# Autodesk Inventor assembly: 2x20ExtraTallHeader
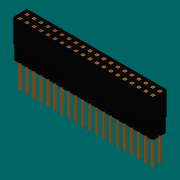
[picture p0: Inventor's stored thumbnail of the model, 180x180]
Saved by Autodesk Inventor 2016 SP1 (Build 200210100, 210)
## iProperties
Created: 2016-04-06
Part Number: 2x20ExtraTallHeader
Document SubType Name: Assembly
Designer: sawai
Author: sawai
## Documents named in this file (2)
- C:\Users\sawai\OneDrive\projects\mppcInterface\cad\connector\2.54Header\piExtraTall\2x20ExtraTallHeader.iam
- C:\Users\sawai\OneDrive\projects\mppcInterface\cad\connector\2.54Header\piExtraTall\extraTallPin.iam
## Components (40 placed, 1 different names)
1. extraTallPin:1 [sub-assembly]
2. extraTallPin:2 [sub-assembly]
3. extraTallPin:3 [sub-assembly]
4. extraTallPin:4 [sub-assembly]
5. extraTallPin:5 [sub-assembly]
6. extraTallPin:6 [sub-assembly]
7. extraTallPin:7 [sub-assembly]
8. extraTallPin:8 [sub-assembly]
9. extraTallPin:9 [sub-assembly]
10. extraTallPin:10 [sub-assembly]
11. extraTallPin:11 [sub-assembly]
12. extraTallPin:12 [sub-assembly]
13. extraTallPin:13 [sub-assembly]
14. extraTallPin:14 [sub-assembly]
15. extraTallPin:15 [sub-assembly]
16. extraTallPin:16 [sub-assembly]
17. extraTallPin:17 [sub-assembly]
18. extraTallPin:18 [sub-assembly]
19. extraTallPin:19 [sub-assembly]
20. extraTallPin:20 [sub-assembly]
21. extraTallPin:21 [sub-assembly]
22. extraTallPin:22 [sub-assembly]
23. extraTallPin:23 [sub-assembly]
24. extraTallPin:24 [sub-assembly]
25. extraTallPin:25 [sub-assembly]
26. extraTallPin:26 [sub-assembly]
27. extraTallPin:27 [sub-assembly]
28. extraTallPin:28 [sub-assembly]
29. extraTallPin:29 [sub-assembly]
30. extraTallPin:30 [sub-assembly]
31. extraTallPin:31 [sub-assembly]
32. extraTallPin:32 [sub-assembly]
33. extraTallPin:33 [sub-assembly]
34. extraTallPin:34 [sub-assembly]
35. extraTallPin:35 [sub-assembly]
36. extraTallPin:36 [sub-assembly]
37. extraTallPin:37 [sub-assembly]
38. extraTallPin:38 [sub-assembly]
39. extraTallPin:39 [sub-assembly]
40. extraTallPin:40 [sub-assembly]
## Component patterns: (40 elements, first: extraTallPin:1)
